# Autodesk Inventor assembly: POM_T5_02
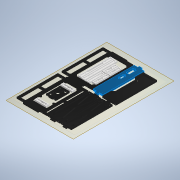
[picture p0: Inventor's stored thumbnail of the model, 180x180]
Saved by Autodesk Inventor 2020 (Build 240168000, 168)
## iProperties
Created: 2021-08-27
Part Number: POM_T5_02
Document SubType Name: Assembly
Designer: Masato
Author: Masato
## Documents named in this file (17)
- C:\Users\naoki\Documents\Inventor\CitBrains\git_clone\SUSTAINA_ver1_0\A_T4_T2\SUSTAINA-OP\Cam\POM_T5_02.iam
- C:\Users\naoki\Documents\Inventor\CitBrains\git_clone\SUSTAINA_ver1_0\A_T4_T2\SUSTAINA-OP\Cam\DisposableBoard.ipt
- C:\Users\naoki\Documents\Inventor\CitBrains\git_clone\SUSTAINA_ver1_0\A_T4_T2\SUSTAINA-OP\UpperBody\Cockpit\Cockpit_carrier_board_frame.ipt
- C:\Users\naoki\Documents\Inventor\CitBrains\git_clone\SUSTAINA_ver1_0\A_T4_T2\SUSTAINA-OP\UpperBody\Cockpit\Cockpit_circuit_board_frame.ipt
- C:\Users\naoki\Documents\Inventor\CitBrains\git_clone\SUSTAINA_ver1_0\A_T4_T2\SUSTAINA-OP\UpperBody\Cockpit\Cockpit_back_frame.ipt
- C:\Users\naoki\Documents\Inventor\CitBrains\git_clone\SUSTAINA_ver1_0\A_T4_T2\SUSTAINA-OP\UpperBody\Cockpit\Cockpit_battery_back_door.ipt
- C:\Users\naoki\Documents\Inventor\CitBrains\git_clone\SUSTAINA_ver1_0\A_T4_T2\SUSTAINA-OP\UpperBody\Cockpit\Cockpit_battery_bottom_frame.ipt
- C:\Users\naoki\Documents\Inventor\CitBrains\git_clone\SUSTAINA_ver1_0\A_T4_T2\SUSTAINA-OP\UpperBody\Cockpit\Cockpit_battery_front_frame.ipt
- C:\Users\naoki\Documents\Inventor\CitBrains\git_clone\SUSTAINA_ver1_0\A_T4_T2\SUSTAINA-OP\Jig\Cockpit_carrier_board_frame_Jig.ipt
- C:\Users\naoki\Documents\Inventor\CitBrains\git_clone\SUSTAINA_ver1_0\A_T4_T2\SUSTAINA-OP\Jig\Cockpit_circuit_board_frame_Jig.ipt
- C:\Users\naoki\Documents\Inventor\CitBrains\git_clone\SUSTAINA_ver1_0\A_T4_T2\SUSTAINA-OP\Jig\Cockpit_battery_back_door_Jig.ipt
- C:\Users\naoki\Documents\Inventor\CitBrains\git_clone\SUSTAINA_ver1_0\A_T4_T2\SUSTAINA-OP\Jig\Cockpit_battery_bottom_frame_Jig.ipt
- C:\Users\naoki\Documents\Inventor\CitBrains\git_clone\SUSTAINA_ver1_0\A_T4_T2\SUSTAINA-OP\Jig\Cockpit_battery_front_frame_Jig.ipt
- C:\Users\naoki\Documents\Inventor\CitBrains\git_clone\SUSTAINA_ver1_0\A_T4_T2\SUSTAINA-OP\Jig\Cockpit_back_frame_Jig.ipt
- C:\Users\naoki\Documents\Inventor\CitBrains\git_clone\SUSTAINA_ver1_0\A_T4_T2\SUSTAINA-OP\Jig\UpperArm_diagonal_Jig.ipt
- C:\Users\naoki\Documents\Inventor\CitBrains\git_clone\SUSTAINA_ver1_0\A_T4_T2\SUSTAINA-OP\UpperBody\Head\Head_horn_frame.ipt
- C:\Users\naoki\Documents\Inventor\CitBrains\git_clone\SUSTAINA_ver1_0\A_T4_T2\SUSTAINA-OP\Jig\Head_horn_frame_Jig.ipt
## Components (16 placed, 16 different names)
1. DisposableBoard:1 — メイト:2, メイト:1, フラッシュ:1, フラッシュ:2, メイト:4, メイト:6, メイト:7, メイト:8, メイト:9, フラッシュ:3, フラッシュ:4, フラッシュ:6, フラッシュ:7, メイト:17, フラッシュ:8, メイト:24, メイト:27, メイト:28, メイト:31, メイト:35, メイト:36, メイト:38, メイト:39, メイト:44
2. Cockpit_carrier_board_frame:1 — メイト:4, フラッシュ:3, フラッシュ:4, メイト:11, メイト:18, メイト:40, メイト:41, メイト:43, メイト:45, メイト:46
3. Cockpit_circuit_board_frame:1 — メイト:17, メイト:18, フラッシュ:8, メイト:19, メイト:25, 正接:2, 正接:3, 正接:4, 正接:5
4. Cockpit_back_frame:1 — メイト:9, メイト:12, メイト:16, メイト:19
5. Cockpit_battery_back_door:1 — メイト:8, メイト:15, メイト:16
6. Cockpit_battery_bottom_frame:1 — メイト:6, フラッシュ:6, メイト:11, メイト:12, メイト:14
7. Cockpit_battery_front_frame:1 — メイト:7, フラッシュ:7, メイト:14, メイト:15
8. Cockpit_battery_back_door_Jig:1 — メイト:24, メイト:25, メイト:29, メイト:34, フラッシュ:9
9. Cockpit_battery_bottom_frame_Jig:1 — メイト:28, メイト:32, 正接:2, メイト:34
10. Cockpit_battery_front_frame_Jig:1 — メイト:27, メイト:29, メイト:33
11. Cockpit_back_frame_Jig:1 — メイト:31, メイト:32, メイト:33
12. Cockpit_carrier_board_frame_Jig:1 — メイト:36, 正接:3, メイト:37, 正接:4, 正接:5
13. Cockpit_circuit_board_frame_Jig:1 — メイト:35, フラッシュ:9, メイト:37
14. UpperArm_diagonal_Jig:1 — メイト:38, メイト:42, メイト:45, メイト:46
15. Head_horn_frame:1 — メイト:42, メイト:43, メイト:44
16. Head_horn_frame_Jig:1 — メイト:39, メイト:40, メイト:41
## Relationships (48: Mate 36, Flush 8, Tangent 4)
- メイト:2 [Mate]: DisposableBoard:1
- メイト:1 [Mate]: DisposableBoard:1
- フラッシュ:1 [Flush]: DisposableBoard:1
- フラッシュ:2 [Flush]: DisposableBoard:1
- メイト:4 [Mate]: DisposableBoard:1 ↔ Cockpit_carrier_board_frame:1
- メイト:6 [Mate]: DisposableBoard:1 ↔ Cockpit_battery_bottom_frame:1
- メイト:7 [Mate]: DisposableBoard:1 ↔ Cockpit_battery_front_frame:1
- メイト:8 [Mate]: DisposableBoard:1 ↔ Cockpit_battery_back_door:1
- メイト:9 [Mate]: DisposableBoard:1 ↔ Cockpit_back_frame:1
- フラッシュ:3 [Flush] (2.5 mm): DisposableBoard:1 ↔ Cockpit_carrier_board_frame:1
- フラッシュ:4 [Flush] (2.5 mm): DisposableBoard:1 ↔ Cockpit_carrier_board_frame:1
- フラッシュ:6 [Flush] (2.5 mm): DisposableBoard:1 ↔ Cockpit_battery_bottom_frame:1
- メイト:11 [Mate] (2.5 mm): Cockpit_carrier_board_frame:1 ↔ Cockpit_battery_bottom_frame:1
- メイト:12 [Mate] (2.5 mm): Cockpit_back_frame:1 ↔ Cockpit_battery_bottom_frame:1
- フラッシュ:7 [Flush] (2.5 mm): DisposableBoard:1 ↔ Cockpit_battery_front_frame:1
- メイト:14 [Mate] (2.5 mm): Cockpit_battery_bottom_frame:1 ↔ Cockpit_battery_front_frame:1
- メイト:15 [Mate] (2.5 mm): Cockpit_battery_back_door:1 ↔ Cockpit_battery_front_frame:1
- メイト:16 [Mate] (2.5 mm): Cockpit_back_frame:1 ↔ Cockpit_battery_back_door:1
- メイト:17 [Mate]: DisposableBoard:1 ↔ Cockpit_circuit_board_frame:1
- メイト:18 [Mate] (2.5 mm): Cockpit_carrier_board_frame:1 ↔ Cockpit_circuit_board_frame:1
- フラッシュ:8 [Flush] (2.5 mm): DisposableBoard:1 ↔ Cockpit_circuit_board_frame:1
- メイト:19 [Mate] (2.5 mm): Cockpit_circuit_board_frame:1 ↔ Cockpit_back_frame:1
- メイト:24 [Mate]: DisposableBoard:1 ↔ Cockpit_battery_back_door_Jig:1
- メイト:25 [Mate] (3 mm): Cockpit_circuit_board_frame:1 ↔ Cockpit_battery_back_door_Jig:1
- メイト:27 [Mate]: DisposableBoard:1 ↔ Cockpit_battery_front_frame_Jig:1
- メイト:28 [Mate]: DisposableBoard:1 ↔ Cockpit_battery_bottom_frame_Jig:1
- メイト:29 [Mate] (2.5 mm): Cockpit_battery_back_door_Jig:1 ↔ Cockpit_battery_front_frame_Jig:1
- メイト:31 [Mate]: DisposableBoard:1 ↔ Cockpit_back_frame_Jig:1
- メイト:32 [Mate] (2.5 mm): Cockpit_battery_bottom_frame_Jig:1 ↔ Cockpit_back_frame_Jig:1
- メイト:33 [Mate] (2.5 mm): Cockpit_battery_front_frame_Jig:1 ↔ Cockpit_back_frame_Jig:1
- 正接:2 [Tangent] (3 mm): Cockpit_circuit_board_frame:1 ↔ Cockpit_battery_bottom_frame_Jig:1
- メイト:34 [Mate] (2.5 mm): Cockpit_battery_back_door_Jig:1 ↔ Cockpit_battery_bottom_frame_Jig:1
- メイト:35 [Mate]: DisposableBoard:1 ↔ Cockpit_circuit_board_frame_Jig:1
- メイト:36 [Mate]: DisposableBoard:1 ↔ Cockpit_carrier_board_frame_Jig:1
- フラッシュ:9 [Flush]: Cockpit_battery_back_door_Jig:1 ↔ Cockpit_circuit_board_frame_Jig:1
- 正接:3 [Tangent] (2.5 mm): Cockpit_circuit_board_frame:1 ↔ Cockpit_carrier_board_frame_Jig:1
- メイト:37 [Mate] (2.5 mm): Cockpit_carrier_board_frame_Jig:1 ↔ Cockpit_circuit_board_frame_Jig:1
- 正接:4 [Tangent] (2.5 mm): Cockpit_circuit_board_frame:1 ↔ Cockpit_carrier_board_frame_Jig:1
- 正接:5 [Tangent] (2.5 mm): Cockpit_circuit_board_frame:1 ↔ Cockpit_carrier_board_frame_Jig:1
- メイト:38 [Mate]: DisposableBoard:1 ↔ UpperArm_diagonal_Jig:1
- メイト:39 [Mate]: DisposableBoard:1 ↔ Head_horn_frame_Jig:1
- メイト:40 [Mate] (2.5 mm): Cockpit_carrier_board_frame:1 ↔ Head_horn_frame_Jig:1
- メイト:41 [Mate] (4 mm): Cockpit_carrier_board_frame:1 ↔ Head_horn_frame_Jig:1
- メイト:42 [Mate] (2.5 mm): UpperArm_diagonal_Jig:1 ↔ Head_horn_frame:1
- メイト:43 [Mate] (7 mm): Cockpit_carrier_board_frame:1 ↔ Head_horn_frame:1
- メイト:44 [Mate]: DisposableBoard:1 ↔ Head_horn_frame:1
- メイト:45 [Mate] (8 mm): Cockpit_carrier_board_frame:1 ↔ UpperArm_diagonal_Jig:1
- メイト:46 [Mate] (4 mm): Cockpit_carrier_board_frame:1 ↔ UpperArm_diagonal_Jig:1
